# Autodesk Inventor assembly: PUERTA SP40-02 INT 2100x800 Doble cristal
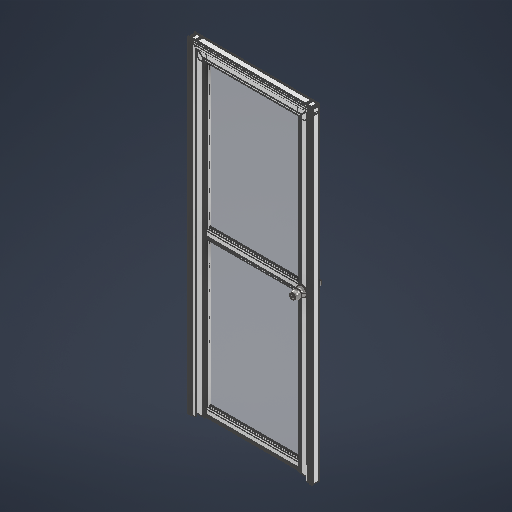
[picture p0: Inventor's stored thumbnail of the model, 512x512]
Saved by Autodesk Inventor 2025 (Build 290162000, 162)
## iProperties
Created: 2026-02-24
Part Number: PUERTA SP40-02 INT 2100x800 Doble cristal
Document SubType Name: Assembly
Designer: ROLANDO
Author: ROLANDO
## Documents named in this file (3)
- C:\Users\rolan\OneDrive\Documentos\Inventor\Projects\CARPINTERIA ALUMINIO\PUERTAS Y VENTANAS\PUERTAS\PUERTAS\PUERTA SP40-02 INT 2100x800 Doble cristal.iam
- C:\Users\rolan\OneDrive\Documentos\Inventor\Projects\CARPINTERIA ALUMINIO\PUERTAS Y VENTANAS\PUERTAS\MARCOS\ENSAMBLES\MARCO SP40-01 2100x800.iam
- C:\Users\rolan\OneDrive\Documentos\Inventor\Projects\CARPINTERIA ALUMINIO\PUERTAS Y VENTANAS\PUERTAS\PUERTAS\ENSAMBLES\PUERTA SP40-02 INT 2100x800 Doble cristal.iam
## Components (2 placed, 2 different names)
1. MARCO SP40-01 2100x800:1 [sub-assembly] — De rotación:1
2. PUERTA SP40-02 INT-EXT 2073x761:1 [sub-assembly] — De rotación:1
## Relationships (1: RevoluteJoint 1)
- De rotación:1 [RevoluteJoint]: MARCO SP40-01 2100x800:1 ↔ PUERTA SP40-02 INT-EXT 2073x761:1
